# Autodesk Inventor assembly: drivetrain
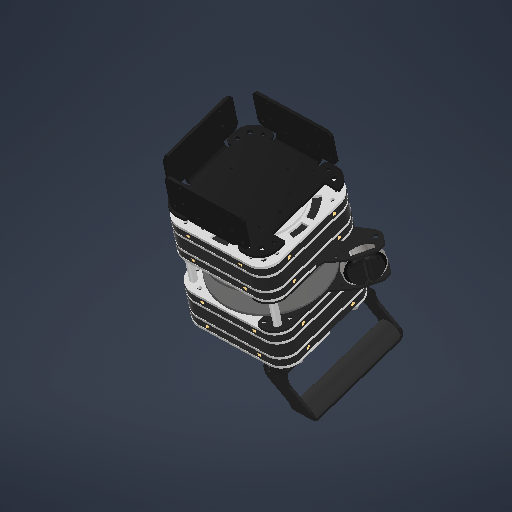
[picture p0: Inventor's stored thumbnail of the model, 512x512]
Saved by Autodesk Inventor 2026.1 (Build 301233000, 233)
## iProperties
Created: 2025-03-02
Part Number: drivetrain
Document SubType Name: Assembly
Designer: aaron
Author: aaron
## Documents named in this file (20)
- D:\work\loopandpixel\openworkoutsystem\cad\v5\drivetrain.iam
- D:\work\loopandpixel\openworkoutsystem\cad\v5\spool.iam
- D:\work\loopandpixel\openworkoutsystem\cad\v5\motor.iam
- D:\work\loopandpixel\openworkoutsystem\cad\v5\shaft_with_keyway.ipt
- D:\work\loopandpixel\openworkoutsystem\cad\v5\M5x40mm_coupler.ipt
- D:\work\loopandpixel\openworkoutsystem\cad\v5\encoder_magnet_holder.ipt
- D:\work\loopandpixel\openworkoutsystem\cad\v5\moteus\20250427-moteus-x1-r1\20250427-moteus-x1-r1\20250427-moteus-x1-r1.ipt
- D:\work\loopandpixel\openworkoutsystem\cad\v5\moteus_x1_mount.ipt
- D:\work\loopandpixel\openworkoutsystem\cad\v5\spool_spacer.ipt
- D:\work\loopandpixel\openworkoutsystem\cad\v5\handle_metal.ipt
- C:\Users\aaron\OneDrive\Documents\Inventor\Content Center Files\R2026\en-US\ANSI B18.3.1M(6)\ANSI B18.3.1M - M5x0.8 x 8(1).ipt
- C:\Users\aaron\OneDrive\Documents\Inventor\Content Center Files\R2026\en-US\ANSI B18.3.1M(6)\ANSI B18.3.1M - M4x0.7 x 6(1).ipt
- D:\work\loopandpixel\openworkoutsystem\cad\v5\handle_insert.ipt
- D:\work\loopandpixel\openworkoutsystem\cad\v5\output_support.ipt
- D:\work\loopandpixel\openworkoutsystem\cad\v5\bearings\bearing_42x30x7.ipt
- C:\Users\aaron\OneDrive\Documents\Inventor\Content Center Files\R2026\en-US\IS 6761\IS 6761 - M3 x 8 - 0.5.ipt
- D:\work\loopandpixel\openworkoutsystem\cad\v5\head_innter_top_42.ipt
- D:\work\loopandpixel\openworkoutsystem\cad\v5\bearings\bearing_12x8x8.ipt
- D:\work\loopandpixel\openworkoutsystem\cad\v5\20250328-x1-heat-spreader\20250328-x1-heat-spreader\20250328-x1-heat-spreader.ipt
- D:\work\loopandpixel\openworkoutsystem\cad\v5\mcthermal_plate.ipt
## Components (37 placed, 19 different names)
1. spool:1 [sub-assembly] — Mate:3, Mate:5, Mate:12
2. motor:2 [sub-assembly] — Mate:1, Mate:4, Insert:22, Flush:1, Mate:6, Flush:2, Mate:11, Flush:4, Flush:5
3. shaft_with_keyway:1 — Mate:2, Mate:3
4. motor:3 [sub-assembly] — Mate:1, Mate:2, Insert:1, Insert:2, Insert:3, Insert:4, Insert:17, Insert:21, Insert:23, Mate:10, Flush:7, Flush:8, Flush:9
5. M5x40mm_coupler:1 — Insert:1, Mate:4
6. M5x40mm_coupler:2 — Insert:3, Mate:19
7. M5x40mm_coupler:3 — Insert:4
8. M5x40mm_coupler:4 — Insert:2
9. encoder_magnet_holder:1 — Insert:17
10. 20250427-moteus-x1-r1:1 — Insert:34, Insert:35, Insert:36, Insert:37
11. moteus_x1_mount:1 — Insert:23, Insert:36, Insert:37
12. spool_spacer:1 — Insert:21, Mate:5
13. spool_spacer:2 — Insert:22, Mate:12
14. handle_metal:1 — Flush:1, Mate:6, Flush:2, Insert:24, Insert:25, Insert:26, Insert:27, Insert:28, Insert:29, Mate:8, Flush:3, Mate:9, Mate:13, Mate:14, Mate:15, Mate:16, Mate:17, Mate:18
15. Forged Socket Head Cap Screw - Metric M5x0.8 x 8:1 — Insert:24
16. Forged Socket Head Cap Screw - Metric M5x0.8 x 8:2 — Insert:25
17. Forged Socket Head Cap Screw - Metric M4x0.7 x 6:1 — Insert:26
18. Forged Socket Head Cap Screw - Metric M4x0.7 x 6:2 — Insert:27
19. Forged Socket Head Cap Screw - Metric M4x0.7 x 6:3 — Insert:28
20. Forged Socket Head Cap Screw - Metric M4x0.7 x 6:4 — Insert:29
21. handle_insert:1 — Mate:8, Flush:3, Mate:9
22. output_support:1 — Mate:10, Flush:6, Flush:7, Mate:20
23. output_support:2 — Mate:11, Flush:4, Flush:5, Mate:20
24. bearing_42x30x7:1 — Flush:6, Insert:30
25. IS 6761 M3 x 8:1 — Mate:13
26. IS 6761 M3 x 8:2 — Mate:14
27. IS 6761 M3 x 8:3 — Mate:15
28. IS 6761 M3 x 8:4 — Mate:16
29. IS 6761 M3 x 8:5 — Mate:17
30. IS 6761 M3 x 8:6 — Mate:18
31. head_innter_top_42:1 — Insert:30
32. bearing_12x8x8:1 — Insert:33
33. bearing_12x8x8:2 — Insert:32, Insert:33
34. bearing_12x8x8:3 — Insert:31, Insert:32
35. bearing_12x8x8:4 — Mate:19, Insert:31
36. 20250328-x1-heat-spreader:1 — Insert:34, Insert:35, Mate:21
37. mcthermal_plate:1 — Flush:8, Flush:9, Mate:21
## Relationships (51: Insert 22, Mate 20, Flush 9)
- Mate:1: motor:2 ↔ motor:3
- Mate:2: shaft_with_keyway:1 ↔ motor:3
- Mate:3: spool:1 ↔ shaft_with_keyway:1
- Insert:1: motor:3 ↔ M5x40mm_coupler:1
- Insert:2: motor:3 ↔ M5x40mm_coupler:4
- Insert:3: motor:3 ↔ M5x40mm_coupler:2
- Insert:4: motor:3 ↔ M5x40mm_coupler:3
- Mate:4: motor:2 ↔ M5x40mm_coupler:1
- Insert:17: motor:3 ↔ encoder_magnet_holder:1
- Insert:21: motor:3 ↔ spool_spacer:1
- Insert:22: motor:2 ↔ spool_spacer:2
- Mate:5: spool:1 ↔ spool_spacer:1
- Insert:23: motor:3 ↔ moteus_x1_mount:1
- Flush:1 (3 mm): motor:2 ↔ handle_metal:1
- Mate:6: motor:2 ↔ handle_metal:1
- Flush:2: motor:2 ↔ handle_metal:1
- Insert:24: handle_metal:1 ↔ Forged Socket Head Cap Screw - Metric M5x0.8 x 8:1
- Insert:25: handle_metal:1 ↔ Forged Socket Head Cap Screw - Metric M5x0.8 x 8:2
- Insert:26: handle_metal:1 ↔ Forged Socket Head Cap Screw - Metric M4x0.7 x 6:1
- Insert:27: handle_metal:1 ↔ Forged Socket Head Cap Screw - Metric M4x0.7 x 6:2
- Insert:28: handle_metal:1 ↔ Forged Socket Head Cap Screw - Metric M4x0.7 x 6:3
- Insert:29: handle_metal:1 ↔ Forged Socket Head Cap Screw - Metric M4x0.7 x 6:4
- Mate:8 (0.2 mm): handle_metal:1 ↔ handle_insert:1
- Flush:3: handle_metal:1 ↔ handle_insert:1
- Mate:9: handle_metal:1 ↔ handle_insert:1
- Mate:10: motor:3 ↔ output_support:1
- Mate:11: motor:2 ↔ output_support:2
- Mate:12: spool:1 ↔ spool_spacer:2
- Flush:4: motor:2 ↔ output_support:2
- Flush:5: motor:2 ↔ output_support:2
- Flush:6 (4 mm): output_support:1 ↔ bearing_42x30x7:1
- Mate:13: handle_metal:1 ↔ IS 6761 M3 x 8:1
- Mate:14: handle_metal:1 ↔ IS 6761 M3 x 8:2
- Mate:15: handle_metal:1 ↔ IS 6761 M3 x 8:3
- Mate:16: handle_metal:1 ↔ IS 6761 M3 x 8:4
- Mate:17: handle_metal:1 ↔ IS 6761 M3 x 8:5
- Mate:18: handle_metal:1 ↔ IS 6761 M3 x 8:6
- Insert:30: bearing_42x30x7:1 ↔ head_innter_top_42:1
- Mate:19: M5x40mm_coupler:2 ↔ bearing_12x8x8:4
- Insert:31: bearing_12x8x8:3 ↔ bearing_12x8x8:4
- Insert:32: bearing_12x8x8:2 ↔ bearing_12x8x8:3
- Insert:33: bearing_12x8x8:1 ↔ bearing_12x8x8:2
- Flush:7: motor:3 ↔ output_support:1
- Mate:20: output_support:1 ↔ output_support:2
- Insert:34: 20250427-moteus-x1-r1:1 ↔ 20250328-x1-heat-spreader:1
- Insert:35: 20250427-moteus-x1-r1:1 ↔ 20250328-x1-heat-spreader:1
- Insert:36: 20250427-moteus-x1-r1:1 ↔ moteus_x1_mount:1
- Insert:37: 20250427-moteus-x1-r1:1 ↔ moteus_x1_mount:1
- Flush:8: motor:3 ↔ mcthermal_plate:1
- Flush:9: motor:3 ↔ mcthermal_plate:1
- Mate:21: 20250328-x1-heat-spreader:1 ↔ mcthermal_plate:1
